# Autodesk Inventor assembly: Сборка5
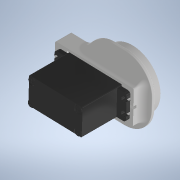
[picture p0: Inventor's stored thumbnail of the model, 180x180]
Saved by Autodesk Inventor 2022 (Build 260153000, 153)
## iProperties
Created: 2023-02-13
Part Number: Сборка5
Document SubType Name: Assembly
Designer: Папа
Author: Папа
## Documents named in this file (4)
- E:\Новая папка\Сборка5.iam
- E:\Новая папка\servoDS3115mg.iam
- E:\Новая папка\DUOPAN-SG.ipt
- E:\Новая папка\мотор_локтя_1.1.ipt
## Components (3 placed, 3 different names)
1. servoDS3115mg:1 [sub-assembly] — Совмещение:1, Совмещение:2, Совмещение:3, Совмещение:4, Совмещение:5
2. DUOPAN-SG:1 — Совмещение:1, Совмещение:2
3. мотор_локтя_1.1:1 — Совмещение:3, Совмещение:4, Совмещение:5
## Relationships (5: Mate 5)
- Совмещение:1 [Mate]: servoDS3115mg:1 ↔ DUOPAN-SG:1
- Совмещение:2 [Mate]: servoDS3115mg:1 ↔ DUOPAN-SG:1
- Совмещение:3 [Mate]: servoDS3115mg:1 ↔ мотор_локтя_1.1:1
- Совмещение:4 [Mate]: servoDS3115mg:1 ↔ мотор_локтя_1.1:1
- Совмещение:5 [Mate]: servoDS3115mg:1 ↔ мотор_локтя_1.1:1
